# Autodesk Inventor assembly: Samolot
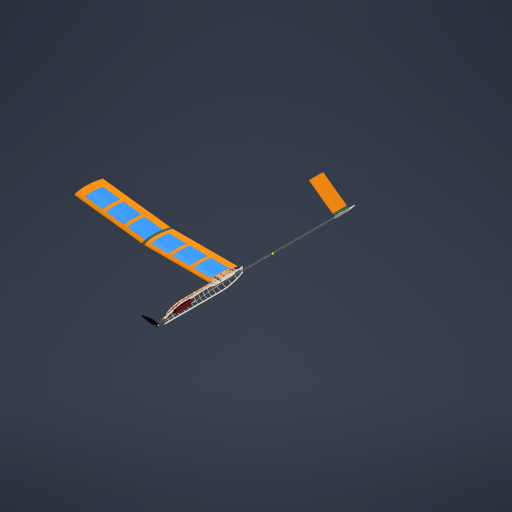
[picture p0: Inventor's stored thumbnail of the model, 512x512]
Saved by Autodesk Inventor 2024 (Build 280153000, 153)
## iProperties
Created: 2023-01-05
Part Number: Samolot
Document SubType Name: Assembly
Designer: szykr
Author: szykr
## Documents named in this file (13)
- C:\Users\Maciej\Desktop\samolot\Solaris\Solaris\new model\Samolot.iam
- C:\Users\Maciej\Desktop\samolot\Solaris\Solaris\new model\Skrzydło.iam
- C:\Users\Maciej\Desktop\samolot\Solaris\Solaris\new model\Tail\Tail.iam
- C:\Users\Maciej\Desktop\samolot\Solaris\Solaris\new model\nowy kadłub.ipt
- C:\Users\Maciej\Desktop\samolot\Solaris\Solaris\new model\Poszycie.ipt
- C:\Users\Maciej\Desktop\samolot\Solaris\Solaris\new model\Poszycie skrzydlo glowne.ipt
- C:\Users\Maciej\Desktop\samolot\Solaris\Solaris\new model\Poszycie skrzydlo sterowe.ipt
- C:\Users\Maciej\Desktop\samolot\Solaris\Solaris\new model\Silnik.ipt
- C:\Users\Maciej\Desktop\samolot\Solaris\Solaris\new model\APC_9x6.ipt
- C:\Users\Maciej\Desktop\samolot\Solaris\Solaris\new model\Panele.ipt
- C:\Users\Maciej\Desktop\samolot\Solaris\Solaris\new model\cienki_spar_dlugi.ipt
- C:\Users\Maciej\Desktop\samolot\Solaris\Solaris\new model\cienki_spar_krotki__ale_troche_dluzszy.ipt
- C:\Users\Maciej\Desktop\samolot\Solaris\Solaris\new model\battery.ipt
## Components (36 placed, 12 different names)
1. Tail:1 [sub-assembly] — Mate:34, Flush:11
2. nowy kadłub:1 — Mate:1, Mate:2, Mate:3, Mate:4, Mate:5, Angle:1, Flush:6, Mate:17, Mate:19, Mate:21, Mate:34, Flush:11, Mate:35
3. Skrzydło:1 [sub-assembly] — Mate:1, Mate:2, Mate:3, Flush:1, Flush:2, Mate:6, Mate:7, Flush:3, Flush:4, Mate:8, Mate:9, Flush:5, Mate:10, Mate:11, Flush:8, Mate:12, Mate:13, Mate:14, Mate:15, Mate:16, Mate:18, Mate:20, Insert:3, Insert:4, Insert:5, Insert:6, Insert:7, Insert:8, Mate:23, Mate:24, Mate:26, Mate:27, Mate:29, Mate:30, Mate:32, Mate:33
4. Poszycie:1 — Mate:4, Mate:5, Angle:1
5. Poszycie skrzydlo glowne:1 — Flush:1, Flush:2
6. Poszycie skrzydlo glowne:2 — Mate:6, Mate:7, Flush:3, Flush:7
7. Poszycie skrzydlo sterowe:1 — Flush:4, Flush:9
8. Poszycie skrzydlo sterowe:2 — Mate:8, Mate:9, Flush:5, Flush:10
9. Silnik:1 — Flush:6, Insert:2
10. APC_9x6:1 — Insert:2
11. cienki_spar_dlugi:1 — Mate:16, Mate:17
12. cienki_spar_dlugi:2 — Mate:18, Mate:19
13. cienki_spar_dlugi:3 — Mate:20, Mate:21, Mate:28, Mate:31
14. cienki_spar_krotki__ale_troche_dluzszy:1 — Insert:3
15. cienki_spar_krotki__ale_troche_dluzszy:2 — Insert:4
16. cienki_spar_krotki__ale_troche_dluzszy:3 — Insert:5, Mate:22
17. cienki_spar_krotki__ale_troche_dluzszy:4 — Insert:8
18. cienki_spar_krotki__ale_troche_dluzszy:5 — Insert:7
19. cienki_spar_krotki__ale_troche_dluzszy:6 — Insert:6, Mate:25
20. Poszycie skrzydlo sterowe:3 — Mate:22, Mate:23, Mate:24
21. Poszycie skrzydlo sterowe:4 — Mate:25, Mate:26, Mate:27
22. Poszycie skrzydlo glowne:3 — Mate:28, Mate:29, Mate:30
23. Poszycie skrzydlo glowne:4 — Mate:31, Mate:32, Mate:33
24. battery:1 — Mate:35
25. Panele:1 — Flush:7
26. Panele:2
27. Panele:3
28. Panele:4 — Mate:10, Mate:11, Flush:8
29. Panele:5
30. Panele:6
31. Panele:7 — Mate:12, Mate:13, Flush:9
32. Panele:8
33. Panele:9
34. Panele:10 — Mate:14, Mate:15, Flush:10
35. Panele:11
36. Panele:12
## Component patterns: (3 elements, first: Panele:1), (3 elements, first: Panele:4), (3 elements, first: Panele:7), (3 elements, first: Panele:10)
## Relationships (54: Mate 35, Flush 11, Insert 7, Angle 1)
- Mate:1: nowy kadłub:1 ↔ Skrzydło:1
- Mate:2: nowy kadłub:1 ↔ Skrzydło:1
- Mate:3: nowy kadłub:1 ↔ Skrzydło:1
- Mate:4: nowy kadłub:1 ↔ Poszycie:1
- Mate:5: nowy kadłub:1 ↔ Poszycie:1
- Angle:1 (180 deg): nowy kadłub:1 ↔ Poszycie:1
- Flush:1: Skrzydło:1 ↔ Poszycie skrzydlo glowne:1
- Flush:2: Skrzydło:1 ↔ Poszycie skrzydlo glowne:1
- Mate:6: Skrzydło:1 ↔ Poszycie skrzydlo glowne:2
- Mate:7: Skrzydło:1 ↔ Poszycie skrzydlo glowne:2
- Flush:3: Skrzydło:1 ↔ Poszycie skrzydlo glowne:2
- Flush:4: Skrzydło:1 ↔ Poszycie skrzydlo sterowe:1
- Mate:8: Skrzydło:1 ↔ Poszycie skrzydlo sterowe:2
- Mate:9: Skrzydło:1 ↔ Poszycie skrzydlo sterowe:2
- Flush:5: Skrzydło:1 ↔ Poszycie skrzydlo sterowe:2
- Flush:6: nowy kadłub:1 ↔ Silnik:1
- Insert:2: Silnik:1 ↔ APC_9x6:1
- Flush:7: Poszycie skrzydlo glowne:2 ↔ Panele:1
- Mate:10: Skrzydło:1 ↔ Panele:4
- Mate:11: Skrzydło:1 ↔ Panele:4
- Flush:8: Skrzydło:1 ↔ Panele:4
- Mate:12: Skrzydło:1 ↔ Panele:7
- Mate:13: Skrzydło:1 ↔ Panele:7
- Flush:9: Poszycie skrzydlo sterowe:1 ↔ Panele:7
- Mate:14: Skrzydło:1 ↔ Panele:10
- Mate:15: Skrzydło:1 ↔ Panele:10
- Flush:10: Poszycie skrzydlo sterowe:2 ↔ Panele:10
- Mate:16: Skrzydło:1 ↔ cienki_spar_dlugi:1
- Mate:17: nowy kadłub:1 ↔ cienki_spar_dlugi:1
- Mate:18: Skrzydło:1 ↔ cienki_spar_dlugi:2
- Mate:19: nowy kadłub:1 ↔ cienki_spar_dlugi:2
- Mate:20: Skrzydło:1 ↔ cienki_spar_dlugi:3
- Mate:21: nowy kadłub:1 ↔ cienki_spar_dlugi:3
- Insert:3: Skrzydło:1 ↔ cienki_spar_krotki__ale_troche_dluzszy:1
- Insert:4: Skrzydło:1 ↔ cienki_spar_krotki__ale_troche_dluzszy:2
- Insert:5: Skrzydło:1 ↔ cienki_spar_krotki__ale_troche_dluzszy:3
- Insert:6: Skrzydło:1 ↔ cienki_spar_krotki__ale_troche_dluzszy:6
- Insert:7: Skrzydło:1 ↔ cienki_spar_krotki__ale_troche_dluzszy:5
- Insert:8: Skrzydło:1 ↔ cienki_spar_krotki__ale_troche_dluzszy:4
- Mate:22: cienki_spar_krotki__ale_troche_dluzszy:3 ↔ Poszycie skrzydlo sterowe:3
- Mate:23: Skrzydło:1 ↔ Poszycie skrzydlo sterowe:3
- Mate:24: Skrzydło:1 ↔ Poszycie skrzydlo sterowe:3
- Mate:25: cienki_spar_krotki__ale_troche_dluzszy:6 ↔ Poszycie skrzydlo sterowe:4
- Mate:26: Skrzydło:1 ↔ Poszycie skrzydlo sterowe:4
- Mate:27: Skrzydło:1 ↔ Poszycie skrzydlo sterowe:4
- Mate:28: cienki_spar_dlugi:3 ↔ Poszycie skrzydlo glowne:3
- Mate:29: Skrzydło:1 ↔ Poszycie skrzydlo glowne:3
- Mate:30: Skrzydło:1 ↔ Poszycie skrzydlo glowne:3
- Mate:31: cienki_spar_dlugi:3 ↔ Poszycie skrzydlo glowne:4
- Mate:32: Skrzydło:1 ↔ Poszycie skrzydlo glowne:4
- Mate:33: Skrzydło:1 ↔ Poszycie skrzydlo glowne:4
- Mate:34: Tail:1 ↔ nowy kadłub:1
- Flush:11: Tail:1 ↔ nowy kadłub:1
- Mate:35: nowy kadłub:1 ↔ battery:1
